# Autodesk Inventor assembly: LongSupportPlateAssembly
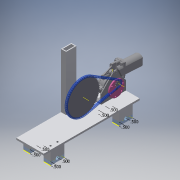
[picture p0: Inventor's stored thumbnail of the model, 180x180]
Saved by Autodesk Inventor 2016 SP1 (Build 200210100, 210)
## iProperties
Created: 2016-02-05
Part Number: LongSupportPlateAssembly
Document SubType Name: Assembly
Designer: steele
Author: steele
## Documents named in this file (6)
- C:\snobotics\CAD-Development\robSteele\SnoBotics2016\2016-01-31-Lift\LongSupportPlateAssembly.iam
- C:\snobotics\CAD-Development\robSteele\SnoBotics2016\2015-02-05-RhinoRobotNarrowView\capForLift.ipt
- C:\snobotics\CAD-Development\robSteele\SnoBotics2016\2016-01-31-Lift\longSupportPlateV02.ipt
- C:\snobotics\CAD-Development\robSteele\SnoBotics2016\AM Parts\SnowBlowerMotorAndHub_MIR.iam
- C:\snobotics\CAD-Development\robSteele\SnoBotics2016\AM Parts\rsSnowBlowerMount.ipt
- C:\snobotics\CAD-Development\robSteele\SnoBotics2016\2016-01-31-Lift\LongSupportPlateAssembly\Design Accelerator\Chain Drive1.iam
## Components (8 placed, 5 different names)
1. longSupportPlateV02:1 — Mate:1, Flush:1, Mate:2, Flush:2, Mate:3, Flush:3, Flush:4, Mate:4, Flush:5, Flush:6, Flush:7, Flush:8, Flush:9, Flush:10, Mate:5, Flush:11, Flush:12
2. capForLift:1 — Mate:1, Flush:1, Flush:8
3. capForLift:2 — Mate:2, Flush:2, Flush:7
4. capForLift:3 — Mate:3, Flush:3, Flush:4, Flush:9
5. capForLift:4 — Mate:4, Flush:5, Flush:6, Flush:10
6. SnowBlowerMotorAndHub_MIR:1 [sub-assembly] — Insert:1
7. rsSnowBlowerMount:2 — Mate:5, Flush:11, Flush:12, Insert:1
8. Chain Drive:1 [sub-assembly]
## Relationships (18: Flush 12, Mate 5, Insert 1)
- Mate:1: longSupportPlateV02:1 ↔ capForLift:1
- Flush:1: longSupportPlateV02:1 ↔ capForLift:1
- Mate:2: longSupportPlateV02:1 ↔ capForLift:2
- Flush:2: longSupportPlateV02:1 ↔ capForLift:2
- Mate:3: longSupportPlateV02:1 ↔ capForLift:3
- Flush:3: longSupportPlateV02:1 ↔ capForLift:3
- Flush:4: longSupportPlateV02:1 ↔ capForLift:3
- Mate:4: longSupportPlateV02:1 ↔ capForLift:4
- Flush:5: longSupportPlateV02:1 ↔ capForLift:4
- Flush:6: longSupportPlateV02:1 ↔ capForLift:4
- Flush:7: longSupportPlateV02:1 ↔ capForLift:2
- Flush:8: longSupportPlateV02:1 ↔ capForLift:1
- Flush:9: longSupportPlateV02:1 ↔ capForLift:3
- Flush:10: longSupportPlateV02:1 ↔ capForLift:4
- Mate:5: longSupportPlateV02:1 ↔ rsSnowBlowerMount:2
- Flush:11 (-50.8 mm): longSupportPlateV02:1 ↔ rsSnowBlowerMount:2
- Flush:12: longSupportPlateV02:1 ↔ rsSnowBlowerMount:2
- Insert:1: SnowBlowerMotorAndHub_MIR:1 ↔ rsSnowBlowerMount:2
